# Autodesk Inventor assembly: Assembly
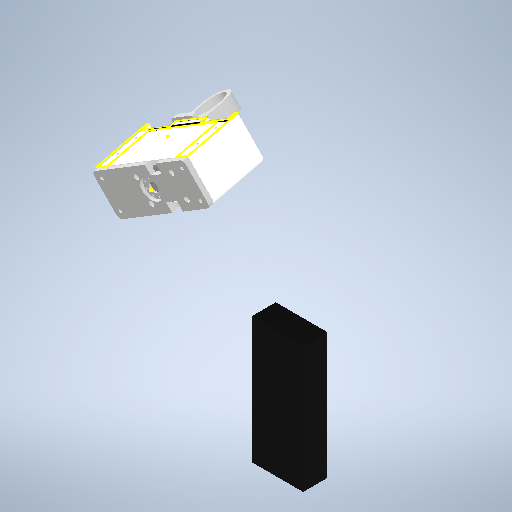
[picture p0: Inventor's stored thumbnail of the model, 512x512]
Saved by Autodesk Inventor 2025.2 (Build 292293000, 293)
## iProperties
Created: 2025-02-13
Part Number: Assembly
Document SubType Name: Assembly
Designer: Admin
Author: Admin
## Documents named in this file (11)
- C:\Users\Admin\Desktop\Masters_Thesis_SDU\exoskeleton\Assembly.iam
- C:\Users\Admin\Desktop\Masters_Thesis_SDU\exoskeleton\guide_cover.ipt
- C:\Users\Admin\Desktop\Masters_Thesis_SDU\exoskeleton\jaw.ipt
- C:\Users\Admin\Downloads\dynamixel-xm430-w350-r-1.snapshot.6\XM430-W350-R\XM430-W350-R\XM430-W350-R.iam
- C:\Users\Admin\Desktop\Masters_Thesis_SDU\exoskeleton\bottom.ipt
- C:\Users\Admin\Desktop\Masters_Thesis_SDU\exoskeleton\main_side.ipt
- C:\Users\Admin\Desktop\Masters_Thesis_SDU\exoskeleton\other_side.ipt
- C:\Users\Admin\Desktop\Masters_Thesis_SDU\exoskeleton\finger_hole_l.ipt
- C:\Users\Admin\Desktop\Masters_Thesis_SDU\exoskeleton\finger_hole_thumb.ipt
- C:\Users\Admin\Downloads\dynamixel-xm430-w350-r-1.snapshot.6\XM430-W350-R\controller_holder.ipt
- C:\Users\Admin\Desktop\Masters_Thesis_SDU\exoskeleton\horn_gear_2.iam
## Components (12 placed, 10 different names)
1. guide_cover:1 — Mate:1, Mate:2, Mate:3, Mate:4, Flush:1
2. jaw:1 — Mate:2, Mate:4, Mate:36, Mate:37, Mate:38
3. jaw:2 — Mate:1, Mate:3, Flush:1, Mate:21, Mate:22, Mate:31, Mate:32, Mate:33, Mate:34
4. XM430-W350-R:1 [sub-assembly] — Mate:19, Mate:20, Mate:23, Mate:39, Mate:40, Mate:41
5. bottom:1 — Mate:19, Mate:20, Mate:23, Flush:3, Mate:30, Mate:41, Mate:42
6. main_side:1 — Mate:24, Mate:25, Mate:26, Flush:3, Mate:27, Mate:28, Mate:29, Mate:30, Mate:35, Mate:42
7. guide_cover:2 — Mate:21, Mate:22, Mate:24, Mate:25, Mate:26
8. other_side:1 — Mate:27, Mate:28, Mate:29, Mate:35
9. finger_hole_l:1 — Mate:31, Mate:32, Mate:33, Mate:34
10. finger_hole_thumb:1 — Mate:36, Mate:37, Mate:38
11. controller_holder:3
12. horn_gear_2:1 [sub-assembly] — Mate:39, Mate:40
## Relationships (30: Mate 28, Flush 2)
- Mate:1: guide_cover:1 ↔ jaw:2
- Mate:2: guide_cover:1 ↔ jaw:1
- Mate:3: guide_cover:1 ↔ jaw:2
- Mate:4: guide_cover:1 ↔ jaw:1
- Flush:1 (-12.5 mm): guide_cover:1 ↔ jaw:2
- Mate:19: XM430-W350-R:1 ↔ bottom:1
- Mate:20: XM430-W350-R:1 ↔ bottom:1
- Mate:21: jaw:2 ↔ guide_cover:2
- Mate:22: jaw:2 ↔ guide_cover:2
- Mate:23: XM430-W350-R:1 ↔ bottom:1
- Mate:24: main_side:1 ↔ guide_cover:2
- Mate:25: main_side:1 ↔ guide_cover:2
- Mate:26: main_side:1 ↔ guide_cover:2
- Flush:3: bottom:1 ↔ main_side:1
- Mate:27: main_side:1 ↔ other_side:1
- Mate:28: main_side:1 ↔ other_side:1
- Mate:29: main_side:1 ↔ other_side:1
- Mate:30: bottom:1 ↔ main_side:1
- Mate:31: jaw:2 ↔ finger_hole_l:1
- Mate:32: jaw:2 ↔ finger_hole_l:1
- Mate:33: jaw:2 ↔ finger_hole_l:1
- Mate:34: jaw:2 ↔ finger_hole_l:1
- Mate:35: main_side:1 ↔ other_side:1
- Mate:36: jaw:1 ↔ finger_hole_thumb:1
- Mate:37: jaw:1 ↔ finger_hole_thumb:1
- Mate:38: jaw:1 ↔ finger_hole_thumb:1
- Mate:39: XM430-W350-R:1 ↔ horn_gear_2:1
- Mate:40: XM430-W350-R:1 ↔ horn_gear_2:1
- Mate:41: XM430-W350-R:1 ↔ bottom:1
- Mate:42: bottom:1 ↔ main_side:1
